# Autodesk Inventor assembly: Сборка сборщика
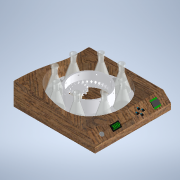
[picture p0: Inventor's stored thumbnail of the model, 180x180]
Saved by Autodesk Inventor 2022 (Build 260153000, 153)
## iProperties
Created: 2022-06-10
Part Number: Сборка сборщика
Document SubType Name: Assembly
Designer: Admin
Author: Admin
## Documents named in this file (16)
- C:\Users\aleks\OneDrive\Рабочий стол\Проект хромотографического сортировщика\Хромотаграфический сборщик модель\Детали\Сборка сборщика.iam
- C:\Users\aleks\OneDrive\Рабочий стол\Проект хромотографического сортировщика\Хромотаграфический сборщик модель\Детали\Барабан.ipt
- C:\Users\aleks\OneDrive\Рабочий стол\Проект хромотографического сортировщика\Хромотаграфический сборщик модель\Детали\короб для подшипника.ipt
- C:\Users\aleks\OneDrive\Рабочий стол\Проект хромотографического сортировщика\Хромотаграфический сборщик модель\Детали\Подшипник.ipt
- C:\Users\aleks\OneDrive\Рабочий стол\Проект хромотографического сортировщика\Хромотаграфический сборщик модель\Детали\штырёк.ipt
- C:\Users\aleks\OneDrive\Рабочий стол\Проект хромотографического сортировщика\Хромотаграфический сборщик модель\Детали\Healical Gear (12R@30.00 m=3.0).ipt
- C:\Users\aleks\OneDrive\Рабочий стол\Проект хромотографического сортировщика\Хромотаграфический сборщик модель\Детали\Healical Gear (32R@30.00 m=3.0).ipt
- C:\Users\aleks\OneDrive\Рабочий стол\Проект хромотографического сортировщика\Хромотаграфический сборщик модель\Детали\Вал.ipt
- C:\Users\aleks\OneDrive\Рабочий стол\Проект хромотографического сортировщика\Хромотаграфический сборщик модель\Детали\Шаговик.ipt
- C:\Users\aleks\OneDrive\Рабочий стол\Проект хромотографического сортировщика\Хромотаграфический сборщик модель\Детали\Кнопка.ipt
- C:\Users\aleks\OneDrive\Рабочий стол\Проект хромотографического сортировщика\Хромотаграфический сборщик модель\Детали\Дисплей.ipt
- C:\Users\aleks\OneDrive\Рабочий стол\Проект хромотографического сортировщика\Хромотаграфический сборщик модель\Детали\Лазер.ipt
- C:\Users\aleks\OneDrive\Рабочий стол\Проект хромотографического сортировщика\Хромотаграфический сборщик модель\Детали\Кнопки на плате.iam
- C:\Users\aleks\OneDrive\Рабочий стол\Проект хромотографического сортировщика\Хромотаграфический сборщик модель\Детали\Измеритель заряда.ipt
- C:\Users\aleks\OneDrive\Рабочий стол\Проект хромотографического сортировщика\Хромотаграфический сборщик модель\Детали\Корпус.ipt
- C:\Users\aleks\OneDrive\Рабочий стол\Проект хромотографического сортировщика\Хромотаграфический сборщик модель\Детали\Колбы\Модель колба коническая 50мл.ipt
## Components (31 placed, 15 different names)
1. Барабан:1 — Совмещение:1, Совмещение:2, Совмещение:3, Совмещение:4, Совмещение:5, Совмещение:6, Совмещение:7, Совмещение:8, Совмещение:14, ЗубчПер:2, С поворотом:11, Совмещение:28, Совмещение:29, Совмещение:30, Совмещение:31, Совмещение:32, Совмещение:33, Совмещение:34, Совмещение:35, Совмещение:36, Совмещение:37, Совмещение:38, Совмещение:39, Совмещение:40, Совмещение:41, Совмещение:42, Совмещение:43, Совмещение:44, Совмещение:45, Совмещение:46, Совмещение:47
2. короб для подшипника:1 — С поворотом:2, Совмещение:3, Совмещение:4, Совмещение:46
3. Подшипник:1 — С поворотом:1
4. штырёк:1 — С поворотом:1, С поворотом:2
5. короб для подшипника:2 — Совмещение:1, Совмещение:2, Совмещение:47, Совмещение:50, Заподлицо:8
6. Подшипник:2 — С поворотом:3
7. штырёк:2 — С поворотом:3, Совмещение:50, Заподлицо:8
8. короб для подшипника:3 — Совмещение:5, Совмещение:6, Совмещение:44, Совмещение:48, Заподлицо:7
9. Подшипник:3 — С поворотом:5
10. штырёк:3 — С поворотом:5, Совмещение:48, Заподлицо:7
11. короб для подшипника:4 — Совмещение:7, Совмещение:8, Совмещение:45, Совмещение:49, Заподлицо:9
12. Подшипник:4 — С поворотом:7
13. штырёк:4 — С поворотом:7, Совмещение:49, Заподлицо:9
14. Healical Gear (12R@30.00 m=3.0):1 — Жесткий:1, Заподлицо:5, ЗубчПер:1
15. Healical Gear (32R@30.00 m=3.0):1 — Заподлицо:5, Совмещение:14, ЗубчПер:1, ЗубчПер:2
16. Вал:1 — С поворотом:10, Жесткий:1
17. Шаговик:1 — С поворотом:10, Совмещение:15, Совмещение:16, Совмещение:17
18. Кнопка:1 — Совмещение:26, Совмещение:27
19. Дисплей:1 — Совмещение:20, Совмещение:21, Совмещение:22
20. Лазер:1 — Жесткий:2
21. Кнопки на плате:1 [sub-assembly] — Совмещение:23, Совмещение:24, Совмещение:25
22. Измеритель заряда:1 — Заподлицо:6, Совмещение:18, Совмещение:19
23. Корпус:1 — С поворотом:11, Совмещение:15, Совмещение:16, Совмещение:17, Заподлицо:6, Совмещение:18, Совмещение:19, Совмещение:20, Совмещение:21, Совмещение:22, Совмещение:23, Совмещение:24, Совмещение:25, Совмещение:26, Совмещение:27, Жесткий:2
24. Модель колба коническая 50мл:1 — Совмещение:28, Совмещение:41
25. Модель колба коническая 50мл:2 — Совмещение:35, Совмещение:42
26. Модель колба коническая 50мл:3 — Совмещение:34, Совмещение:43
27. Модель колба коническая 50мл:4 — Совмещение:33, Совмещение:36
28. Модель колба коническая 50мл:5 — Совмещение:32, Совмещение:37
29. Модель колба коническая 50мл:6 — Совмещение:31, Совмещение:38
30. Модель колба коническая 50мл:7 — Совмещение:30, Совмещение:40
31. Модель колба коническая 50мл:8 — Совмещение:29, Совмещение:39
## Relationships (61: Mate 45, RevoluteJoint 7, Flush 5, WeldJoint 2, RelateRotation 2)
- С поворотом:1 [RevoluteJoint]: Подшипник:1 ↔ штырёк:1
- С поворотом:2 [RevoluteJoint]: короб для подшипника:1 ↔ штырёк:1
- С поворотом:3 [RevoluteJoint]: Подшипник:2 ↔ штырёк:2
- С поворотом:5 [RevoluteJoint]: Подшипник:3 ↔ штырёк:3
- С поворотом:7 [RevoluteJoint]: Подшипник:4 ↔ штырёк:4
- Совмещение:1 [Mate] (0.1 mm): Барабан:1 ↔ короб для подшипника:2
- Совмещение:2 [Mate] (0.1 mm): Барабан:1 ↔ короб для подшипника:2
- Совмещение:3 [Mate] (0.1 mm): Барабан:1 ↔ короб для подшипника:1
- Совмещение:4 [Mate] (0.1 mm): Барабан:1 ↔ короб для подшипника:1
- Совмещение:5 [Mate] (0.1 mm): Барабан:1 ↔ короб для подшипника:3
- Совмещение:6 [Mate] (0.1 mm): Барабан:1 ↔ короб для подшипника:3
- Совмещение:7 [Mate] (0.1 mm): Барабан:1 ↔ короб для подшипника:4
- Совмещение:8 [Mate] (0.1 mm): Барабан:1 ↔ короб для подшипника:4
- С поворотом:10 [RevoluteJoint]: Вал:1 ↔ Шаговик:1
- Жесткий:1 [WeldJoint]: Healical Gear (12R@30.00 m=3.0):1 ↔ Вал:1
- Заподлицо:5 [Flush]: Healical Gear (12R@30.00 m=3.0):1 ↔ Healical Gear (32R@30.00 m=3.0):1
- Совмещение:14 [Mate]: Барабан:1 ↔ Healical Gear (32R@30.00 m=3.0):1
- ЗубчПер:1 [RelateRotation] (0.375 ul): Healical Gear (12R@30.00 m=3.0):1 ↔ Healical Gear (32R@30.00 m=3.0):1
- ЗубчПер:2 [RelateRotation] (1 ul): Барабан:1 ↔ Healical Gear (32R@30.00 m=3.0):1
- С поворотом:11 [RevoluteJoint] (7.359 mm): Барабан:1 ↔ Корпус:1
- Совмещение:15 [Mate]: Шаговик:1 ↔ Корпус:1
- Совмещение:16 [Mate]: Шаговик:1 ↔ Корпус:1
- Совмещение:17 [Mate]: Шаговик:1 ↔ Корпус:1
- Заподлицо:6 [Flush]: Измеритель заряда:1 ↔ Корпус:1
- Совмещение:18 [Mate]: Измеритель заряда:1 ↔ Корпус:1
- Совмещение:19 [Mate]: Измеритель заряда:1 ↔ Корпус:1
- Совмещение:20 [Mate]: Дисплей:1 ↔ Корпус:1
- Совмещение:21 [Mate]: Дисплей:1 ↔ Корпус:1
- Совмещение:22 [Mate] (0.1 mm): Дисплей:1 ↔ Корпус:1
- Совмещение:23 [Mate]: Кнопки на плате:1 ↔ Корпус:1
- Совмещение:24 [Mate]: Кнопки на плате:1 ↔ Корпус:1
- Совмещение:25 [Mate]: Кнопки на плате:1 ↔ Корпус:1
- Совмещение:26 [Mate]: Кнопка:1 ↔ Корпус:1
- Совмещение:27 [Mate]: Кнопка:1 ↔ Корпус:1
- Жесткий:2 [WeldJoint]: Лазер:1 ↔ Корпус:1
- Совмещение:28 [Mate]: Барабан:1 ↔ Модель колба коническая 50мл:1
- Совмещение:29 [Mate]: Барабан:1 ↔ Модель колба коническая 50мл:8
- Совмещение:30 [Mate]: Барабан:1 ↔ Модель колба коническая 50мл:7
- Совмещение:31 [Mate]: Барабан:1 ↔ Модель колба коническая 50мл:6
- Совмещение:32 [Mate]: Барабан:1 ↔ Модель колба коническая 50мл:5
- Совмещение:33 [Mate]: Барабан:1 ↔ Модель колба коническая 50мл:4
- Совмещение:34 [Mate]: Барабан:1 ↔ Модель колба коническая 50мл:3
- Совмещение:35 [Mate]: Барабан:1 ↔ Модель колба коническая 50мл:2
- Совмещение:36 [Mate]: Барабан:1 ↔ Модель колба коническая 50мл:4
- Совмещение:37 [Mate]: Барабан:1 ↔ Модель колба коническая 50мл:5
- Совмещение:38 [Mate]: Барабан:1 ↔ Модель колба коническая 50мл:6
- Совмещение:39 [Mate]: Барабан:1 ↔ Модель колба коническая 50мл:8
- Совмещение:40 [Mate]: Барабан:1 ↔ Модель колба коническая 50мл:7
- Совмещение:41 [Mate]: Барабан:1 ↔ Модель колба коническая 50мл:1
- Совмещение:42 [Mate]: Барабан:1 ↔ Модель колба коническая 50мл:2
- Совмещение:43 [Mate]: Барабан:1 ↔ Модель колба коническая 50мл:3
- Совмещение:44 [Mate]: Барабан:1 ↔ короб для подшипника:3
- Совмещение:45 [Mate]: Барабан:1 ↔ короб для подшипника:4
- Совмещение:46 [Mate]: Барабан:1 ↔ короб для подшипника:1
- Совмещение:47 [Mate]: Барабан:1 ↔ короб для подшипника:2
- Совмещение:48 [Mate]: короб для подшипника:3 ↔ штырёк:3
- Совмещение:49 [Mate]: короб для подшипника:4 ↔ штырёк:4
- Совмещение:50 [Mate]: короб для подшипника:2 ↔ штырёк:2
- Заподлицо:7 [Flush]: короб для подшипника:3 ↔ штырёк:3
- Заподлицо:8 [Flush]: короб для подшипника:2 ↔ штырёк:2
- Заподлицо:9 [Flush]: короб для подшипника:4 ↔ штырёк:4
